# Autodesk Inventor assembly: center-machine-assembly
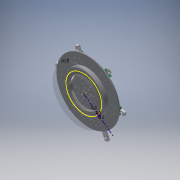
[picture p0: Inventor's stored thumbnail of the model, 180x180]
Saved by Autodesk Inventor 2018 (Build 220112000, 112)
## iProperties
Created: 2025-02-24
Part Number: center-machine-assembly
Document SubType Name: Assembly
Designer: neo
Author: neo
## Documents named in this file (8)
- C:\Users\neo\Documents\projects\kreion\design1\center-machine-assembly.iam
- C:\Users\neo\Documents\projects\kreion\design1\bearing100-80-10.ipt
- C:\Users\neo\Documents\projects\kreion\design1\bearing-base-lower-case.ipt
- C:\Users\neo\Documents\projects\kreion\design1\bearing-base-uppercase.ipt
- C:\Users\neo\Documents\projects\kreion\design1\piston-star-connector.ipt
- C:\Users\neo\Documents\projects\kreion\design1\rotor-case.ipt
- C:\Users\neo\Documents\projects\kreion\design1\slider.iam
- C:\Users\neo\Documents\projects\kreion\design1\magnet-holder.ipt
## Components (12 placed, 7 different names)
1. bearing100-80-10:1 — Tangent:1, Mate:1, Tangent:2, Mate:2, Mate:3, Tangent:4
2. bearing-base-lower-case:1 — Tangent:1, Mate:1, Tangent:3
3. bearing-base-uppercase:1 — Tangent:2, Mate:2, Tangent:3, Mate:5
4. piston-star-connector:1
5. rotor-case:1 — Mate:3, Tangent:4, Mate:6, Mate:7, Tangent:5, Tangent:6, Mate:8, Mate:9, Mate:10, Mate:11, Tangent:7, Tangent:8, Mate:12, Tangent:9, Tangent:10, Tangent:11, Tangent:12, Tangent:13, Tangent:14, Tangent:15, Tangent:16
6. slider:1 [sub-assembly] — Mate:7, Tangent:5, Tangent:6
7. slider:2 [sub-assembly] — Mate:8, Tangent:7, Tangent:8, Flush:1, Mate:13, Tangent:17
8. slider:3 [sub-assembly] — Mate:9, Tangent:15, Tangent:16
9. slider:4 [sub-assembly] — Mate:10, Tangent:13, Tangent:14
10. slider:5 [sub-assembly] — Mate:12, Tangent:9, Tangent:10
11. slider:6 [sub-assembly] — Mate:11, Tangent:11, Tangent:12
12. magnet-holder:1 — Flush:1, Mate:13, Tangent:17
## Relationships (30: Tangent 17, Mate 12, Flush 1)
- Tangent:1: bearing100-80-10:1 ↔ bearing-base-lower-case:1
- Mate:1: bearing100-80-10:1 ↔ bearing-base-lower-case:1
- Tangent:2: bearing100-80-10:1 ↔ bearing-base-uppercase:1
- Mate:2: bearing100-80-10:1 ↔ bearing-base-uppercase:1
- Tangent:3: bearing-base-lower-case:1 ↔ bearing-base-uppercase:1
- Mate:3: bearing100-80-10:1 ↔ rotor-case:1
- Tangent:4: bearing100-80-10:1 ↔ rotor-case:1
- Mate:5: bearing-base-uppercase:1
- Mate:6: rotor-case:1
- Mate:7: rotor-case:1 ↔ slider:1
- Tangent:5: rotor-case:1 ↔ slider:1
- Tangent:6: rotor-case:1 ↔ slider:1
- Mate:8: rotor-case:1 ↔ slider:2
- Mate:9: rotor-case:1 ↔ slider:3
- Mate:10: rotor-case:1 ↔ slider:4
- Mate:11: rotor-case:1 ↔ slider:6
- Tangent:7: rotor-case:1 ↔ slider:2
- Tangent:8: rotor-case:1 ↔ slider:2
- Mate:12: rotor-case:1 ↔ slider:5
- Tangent:9: rotor-case:1 ↔ slider:5
- Tangent:10: rotor-case:1 ↔ slider:5
- Tangent:11: rotor-case:1 ↔ slider:6
- Tangent:12: rotor-case:1 ↔ slider:6
- Tangent:13: rotor-case:1 ↔ slider:4
- Tangent:14: rotor-case:1 ↔ slider:4
- Tangent:15: rotor-case:1 ↔ slider:3
- Tangent:16: rotor-case:1 ↔ slider:3
- Flush:1: slider:2 ↔ magnet-holder:1
- Mate:13: slider:2 ↔ magnet-holder:1
- Tangent:17: slider:2 ↔ magnet-holder:1
